# Autodesk Inventor assembly: socket
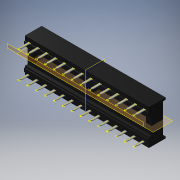
[picture p0: Inventor's stored thumbnail of the model, 180x180]
Saved by Autodesk Inventor 2018 (Build 220112000, 112)
## iProperties
Created: 2017-04-13
Part Number: socket
Document SubType Name: Assembly
Designer: kampe_000
Author: kampe_000
## Documents named in this file (3)
- D:\Kod\stepCounter\CAD\Inventor Project\assembly\socket.iam
- D:\Kod\stepCounter\CAD\Inventor Project\parts\socket.ipt
- D:\Kod\stepCounter\CAD\Inventor Project\parts\socket_pin.ipt
## Components (29 placed, 2 different names)
1. socket:1 — Mate:1, Mate:2, Mate:3
2. socket_pin:1 — Mate:1, Mate:2, Mate:3
3. socket_pin:2
4. socket_pin:3
5. socket_pin:4
6. socket_pin:5
7. socket_pin:6
8. socket_pin:7
9. socket_pin:8
10. socket_pin:9
11. socket_pin:10
12. socket_pin:11
13. socket_pin:12
14. socket_pin:13
15. socket_pin:14
16. socket_pin:15
17. socket_pin:16
18. socket_pin:17
19. socket_pin:18
20. socket_pin:19
21. socket_pin:20
22. socket_pin:21
23. socket_pin:22
24. socket_pin:23
25. socket_pin:24
26. socket_pin:25
27. socket_pin:26
28. socket_pin:27
29. socket_pin:28
## Component patterns: (28 elements, first: socket_pin:1)
## Relationships (3: Mate 3)
- Mate:1: socket:1 ↔ socket_pin:1
- Mate:2: socket:1 ↔ socket_pin:1
- Mate:3: socket:1 ↔ socket_pin:1
